# Autodesk Inventor assembly: aircilinder_60
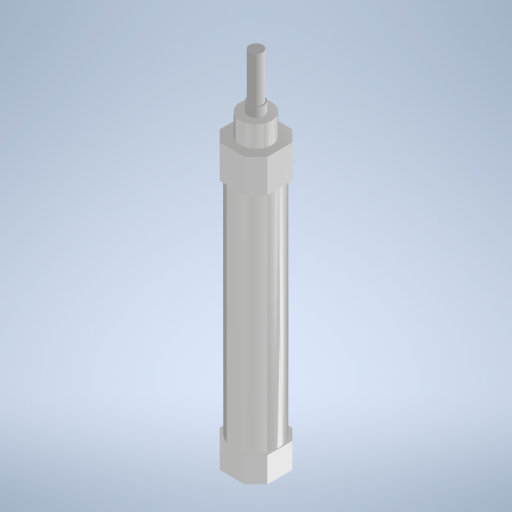
[picture p0: Inventor's stored thumbnail of the model, 512x512]
Saved by Autodesk Inventor 2024.1 (Build 281209000, 209)
## iProperties
Created: 2022-08-24
Part Number: aircilinder_60
Document SubType Name: Assembly
Designer: zegi
Author: zegi
## Documents named in this file (3)
- C:\Users\haruy\OneDrive - Kyushu University\KURT_工房共有\2023~2024\ハード\CAD\2024NHK\000_parts\エアシリンダー\airclinder\aircilinder_60.iam
- C:\Users\haruy\OneDrive - Kyushu University\KURT_工房共有\2023~2024\ハード\CAD\2024NHK\000_parts\エアシリンダー\airclinder\aircilinder_60_lod.ipt
- C:\Users\haruy\OneDrive - Kyushu University\KURT_工房共有\2023~2024\ハード\CAD\2024NHK\000_parts\エアシリンダー\airclinder\airclinder_60.ipt
## Components (2 placed, 2 different names)
1. aircilinder_60_lod:1 — 円柱状:1
2. airclinder_60:1 — 円柱状:1
## Relationships (1: CylindricalJoint 1)
- 円柱状:1 [CylindricalJoint]: aircilinder_60_lod:1 ↔ airclinder_60:1
